# Autodesk Inventor assembly: ball caster model
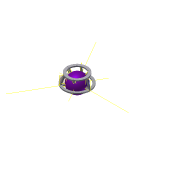
[picture p0: Inventor's stored thumbnail of the model, 180x180]
Saved by Autodesk Inventor 2012 (Build 160160000, 160)
## iProperties
Created: 2011-10-07
Part Number: ball caster model
Document SubType Name: Assembly
Designer: Antonella
Author: Antonella
## Documents named in this file (8)
- C:\Users\Antonella\Documents\GCC Robotics 2012 - Mechanical\Robot 2.0\Ball Caster\ball caster.iam
- C:\Users\Antonella\Documents\GCC Robotics 2012 - Mechanical\Robot 2.0\Ball Caster\ball model.ipt
- C:\Users\Antonella\Documents\GCC Robotics 2012 - Mechanical\Robot 2.0\Ball Caster\ring_top.ipt
- C:\Users\Antonella\Documents\GCC Robotics 2012 - Mechanical\Robot 2.0\Ball Caster\ring_middle.ipt
- C:\Users\Antonella\Documents\GCC Robotics 2012 - Mechanical\Robot 2.0\Ball Caster\ball_transfer.iam
- C:\Users\Antonella\Documents\GCC Robotics 2012 - Mechanical\Robot 2.0\Ball Caster\transfer mount block.ipt
- C:\Users\Antonella\Documents\GCC Robotics 2012 - Mechanical\Robot 2.0\Ball Caster\wedge mount.ipt
- C:\Users\Antonella\Documents\GCC Robotics 2012 - Mechanical\Robot 2.0\Ball Caster\brace.ipt
## Components (16 placed, 7 different names)
1. ball model:1 — Mate:1, Flush:1, Flush:2, Mate:2, Mate:3, Tangent:1, Tangent:2, Tangent:3, Tangent:4
2. ring_top:1 — Mate:2, Mate:3, Mate:11, Mate:12, Mate:13, Mate:14, Mate:15, Mate:16, Mate:17, Mate:18, Mate:19, Mate:26, Mate:27, Tangent:5, Mate:28, Tangent:6, Mate:30, Tangent:7, Mate:32, Tangent:8
3. ring_middle:1 — Mate:1, Flush:1, Flush:2, Mate:4, Mate:5, Mate:6, Mate:29, Mate:31, Mate:33
4. ball_transfer:1 [sub-assembly] — Mate:4, Tangent:3
5. ball_transfer:2 [sub-assembly] — Mate:6, Tangent:1
6. ball_transfer:3 [sub-assembly] — Mate:5, Tangent:2
7. transfer mount block:1 — Mate:14, Mate:15, Mate:16, Mate:20, Mate:21
8. transfer mount block:2 — Mate:11, Mate:12, Mate:13, Mate:22, Mate:23
9. transfer mount block:3 — Mate:17, Mate:18, Mate:19, Mate:24, Mate:25
10. ball_transfer:4 [sub-assembly] — Mate:20, Mate:21, Tangent:4
11. ball_transfer:5 [sub-assembly] — Mate:22, Mate:23
12. ball_transfer:6 [sub-assembly] — Mate:24, Mate:25
13. wedge mount:1 — Mate:26, Mate:27, Tangent:5
14. brace:1 — Mate:28, Tangent:6, Mate:29
15. brace:2 — Mate:32, Mate:33, Tangent:8
16. brace:3 — Mate:30, Tangent:7, Mate:31
## Relationships (39: Mate 29, Tangent 8, Flush 2)
- Mate:1: ball model:1 ↔ ring_middle:1
- Flush:1: ball model:1 ↔ ring_middle:1
- Flush:2: ball model:1 ↔ ring_middle:1
- Mate:2: ball model:1 ↔ ring_top:1
- Mate:3: ball model:1 ↔ ring_top:1
- Mate:4: ring_middle:1 ↔ ball_transfer:1
- Mate:5: ring_middle:1 ↔ ball_transfer:3
- Mate:6: ring_middle:1 ↔ ball_transfer:2
- Tangent:1: ball model:1 ↔ ball_transfer:2
- Tangent:2: ball model:1 ↔ ball_transfer:3
- Tangent:3: ball model:1 ↔ ball_transfer:1
- Mate:11: ring_top:1 ↔ transfer mount block:2
- Mate:12: ring_top:1 ↔ transfer mount block:2
- Mate:13: ring_top:1 ↔ transfer mount block:2
- Mate:14: ring_top:1 ↔ transfer mount block:1
- Mate:15: ring_top:1 ↔ transfer mount block:1
- Mate:16: ring_top:1 ↔ transfer mount block:1
- Mate:17: ring_top:1 ↔ transfer mount block:3
- Mate:18: ring_top:1 ↔ transfer mount block:3
- Mate:19: ring_top:1 ↔ transfer mount block:3
- Mate:20: transfer mount block:1 ↔ ball_transfer:4
- Mate:21: transfer mount block:1 ↔ ball_transfer:4
- Mate:22: transfer mount block:2 ↔ ball_transfer:5
- Mate:23: transfer mount block:2 ↔ ball_transfer:5
- Mate:24: transfer mount block:3 ↔ ball_transfer:6
- Mate:25: transfer mount block:3 ↔ ball_transfer:6
- Tangent:4: ball model:1 ↔ ball_transfer:4
- Mate:26: ring_top:1 ↔ wedge mount:1
- Mate:27: ring_top:1 ↔ wedge mount:1
- Tangent:5: ring_top:1 ↔ wedge mount:1
- Mate:28: ring_top:1 ↔ brace:1
- Tangent:6: ring_top:1 ↔ brace:1
- Mate:29: ring_middle:1 ↔ brace:1
- Mate:30: ring_top:1 ↔ brace:3
- Tangent:7: ring_top:1 ↔ brace:3
- Mate:31: ring_middle:1 ↔ brace:3
- Mate:32: ring_top:1 ↔ brace:2
- Mate:33: ring_middle:1 ↔ brace:2
- Tangent:8: ring_top:1 ↔ brace:2
